# Autodesk Inventor assembly: engranajes motor hombro dimer 3.1_MIR
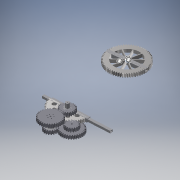
[picture p0: Inventor's stored thumbnail of the model, 180x180]
Saved by Autodesk Inventor 2016 (Build 200138000, 138)
## iProperties
Created: 2016-06-23
Part Number: engranajes motor hombro dimer 3.1_MIR
Document SubType Name: Assembly
Designer: Admin
Author: Admin
## Documents named in this file (12)
- C:\Users\Admin\Documents\diseños autodesk dimer\engranajes dimer hombro muelles\engranajes motor hombro dimer 3.1_MIR.iam
- C:\Users\Admin\Documents\piezas 3d dimer\engranajes motor hombro dimer 3.1\Design Accelerator\Spur Gears1_MIR.iam
- C:\Users\Admin\Documents\piezas 3d dimer\engranajes motor hombro dimer 3.1\Design Accelerator\Spur Gears3_MIR.iam
- C:\Users\Admin\Documents\diseños autodesk dimer\engranajes dimer hombro muelles\perfil aluminio_MIR.ipt
- C:\Users\Admin\Documents\diseños autodesk dimer\engranajes dimer hombro muelles\caja perfil_MIR.ipt
- C:\Users\Admin\Documents\diseños autodesk dimer\engranajes dimer hombro muelles\eje motor_MIR.ipt
- C:\Users\Admin\Documents\diseños autodesk dimer\engranajes dimer hombro muelles\engranajes motor hombro dimer 3.1\Design Accelerator\Spur Gears1_MIR.iam
- C:\Users\Admin\Documents\diseños autodesk dimer\engranajes dimer hombro muelles\engranajes motor hombro dimer 3.1\Design Accelerator\Spur Gears2_MIR.iam
- C:\Users\Admin\Documents\diseños autodesk dimer\engranajes dimer hombro muelles\eje union engrane reductor_MIR.ipt
- C:\Users\Admin\Documents\diseños autodesk dimer\engranajes dimer hombro muelles\engranajes motor hombro dimer 3.1\Design Accelerator\Spur Gear11_MIR.ipt
- C:\Users\Admin\Documents\piezas 3d dimer\engranajes motor hombro dimer 3.1\Design Accelerator\Spur Gear23_MIR.ipt
- C:\Users\Admin\Documents\diseños autodesk dimer\engranajes dimer hombro muelles\engranaje gusano_MIR.ipt
## Components (13 placed, 10 different names)
1. Spur Gears1_MIR:1 [sub-assembly] — Flush:7, Mate:4, Mate:9, Rotation:1, Tangent:1
2. Spur Gears3_MIR:1 [sub-assembly] — Flush:3, Mate:2, Flush:9
3. perfil aluminio_MIR:1 — Flush:6, Flush:5, Flush:4, Mate:12
4. caja perfil_MIR:1 — Flush:6, Flush:5, Flush:4, Flush:3, Mate:2
5. eje motor_MIR:1 — Flush:7, Mate:4
6. Spur Gears1_MIR:2 [sub-assembly] — Mate:9, Rotation:1, Tangent:1, Mate:6, Mate:5, Mate:7
7. Spur Gears2_MIR:1 [sub-assembly] — Mate:6, Mate:5, Mate:8, Flush:8
8. eje union engrane reductor_MIR:1 — Mate:8, Mate:7
9. Spur Gear11_MIR:1 — Flush:8, Mate:11, Mate:10
10. Spur Gears2_MIR:2 [sub-assembly] — Flush:9, Mate:11, Mate:10
11. Spur Gear23_MIR:1 — Mate:12, Flush:15, Flush:14
12. caja perfil_MIR:2 — Flush:15, Flush:14
13. engranaje gusano_MIR:1
## Relationships (21: Mate 10, Flush 9, RelateRotation 1, Tangent 1)
- Flush:6 (-100 mm): perfil aluminio_MIR:1 ↔ caja perfil_MIR:1
- Flush:5 (2.5 mm): perfil aluminio_MIR:1 ↔ caja perfil_MIR:1
- Flush:4 (2.5 mm): perfil aluminio_MIR:1 ↔ caja perfil_MIR:1
- Flush:3: Spur Gears3_MIR:1 ↔ caja perfil_MIR:1
- Mate:2 (-8.5 mm): Spur Gears3_MIR:1 ↔ caja perfil_MIR:1
- Flush:7: Spur Gears1_MIR:1 ↔ eje motor_MIR:1
- Mate:4: Spur Gears1_MIR:1 ↔ eje motor_MIR:1
- Mate:9 (-15 mm): Spur Gears1_MIR:1 ↔ Spur Gears1_MIR:2
- Rotation:1 [RelateRotation] (1 ul): Spur Gears1_MIR:1 ↔ Spur Gears1_MIR:2
- Tangent:1: Spur Gears1_MIR:1 ↔ Spur Gears1_MIR:2
- Mate:6 (26 mm): Spur Gears1_MIR:2 ↔ Spur Gears2_MIR:1
- Mate:5: Spur Gears1_MIR:2 ↔ Spur Gears2_MIR:1
- Mate:8: Spur Gears2_MIR:1 ↔ eje union engrane reductor_MIR:1
- Mate:7: Spur Gears1_MIR:2 ↔ eje union engrane reductor_MIR:1
- Flush:8: Spur Gears2_MIR:1 ↔ Spur Gear11_MIR:1
- Flush:9: Spur Gears3_MIR:1 ↔ Spur Gears2_MIR:2
- Mate:11: Spur Gear11_MIR:1 ↔ Spur Gears2_MIR:2
- Mate:10: Spur Gear11_MIR:1 ↔ Spur Gears2_MIR:2
- Mate:12 (250 mm): perfil aluminio_MIR:1 ↔ Spur Gear23_MIR:1
- Flush:15 (-6 mm): Spur Gear23_MIR:1 ↔ caja perfil_MIR:2
- Flush:14: Spur Gear23_MIR:1 ↔ caja perfil_MIR:2
